# Autodesk Inventor assembly: Pusher2
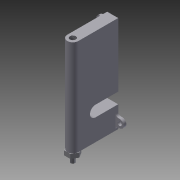
[picture p0: Inventor's stored thumbnail of the model, 180x180]
Saved by Autodesk Inventor 2011 (Build 150239000, 239)
## iProperties
Created: 2011-04-12
Part Number: Pusher2
Document SubType Name: Assembly
Designer: Rob
Author: Rob
## Documents named in this file (5)
- C:\Users\M. Woods III\Desktop\design\Mechanical Drawings\pusher_2.iam
- C:\Users\M. Woods III\Desktop\design\Mechanical Drawings\pusher_2_holder.ipt
- C:\Users\M. Woods III\Desktop\design\Mechanical Drawings\pusher_springplate.ipt
- C:\Users\M. Woods III\Desktop\design\Mechanical Drawings\pusher_bolt.ipt
- C:\Users\M. Woods III\Desktop\design\Mechanical Drawings\pusher_pushrod.ipt
## Components (6 placed, 4 different names)
1. pusher_2_holder:1 — Flush:1, Mate:1, Flush:2, Mate:2, Flush:3, Mate:3, Mate:4, Mate:5, Mate:8
2. pusher_springplate:2 — Flush:3, Mate:3
3. pusher_springplate:3 — Flush:2, Mate:2
4. pusher_springplate:4 — Flush:1, Mate:1
5. pusher_bolt:1 — Mate:4, Mate:5, Mate:7, Flush:4
6. pusher_pushrod:1 — Mate:7, Mate:8, Flush:4
## Relationships (11: Mate 7, Flush 4)
- Flush:1 (9.603 mm): pusher_2_holder:1 ↔ pusher_springplate:4
- Mate:1: pusher_2_holder:1 ↔ pusher_springplate:4
- Flush:2 (44.512 mm): pusher_2_holder:1 ↔ pusher_springplate:3
- Mate:2: pusher_2_holder:1 ↔ pusher_springplate:3
- Flush:3 (79.412 mm): pusher_2_holder:1 ↔ pusher_springplate:2
- Mate:3: pusher_2_holder:1 ↔ pusher_springplate:2
- Mate:4: pusher_2_holder:1 ↔ pusher_bolt:1
- Mate:5: pusher_2_holder:1 ↔ pusher_bolt:1
- Mate:7: pusher_bolt:1 ↔ pusher_pushrod:1
- Mate:8: pusher_2_holder:1 ↔ pusher_pushrod:1
- Flush:4 (-10 mm): pusher_bolt:1 ↔ pusher_pushrod:1
